# Autodesk Inventor assembly: MIR_HbHand
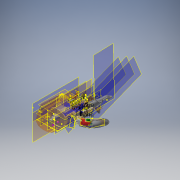
[picture p0: Inventor's stored thumbnail of the model, 180x180]
Saved by Autodesk Inventor 2017 (Build 210142000, 142)
## iProperties
Part Number: MIR_HbHand
Material: 一般
Document SubType Name: Assembly
Designer: sktom
Author: sktom
## Documents named in this file (36)
- D:\OneDrive\CAD\MAJ\hackberry\HACKberry-hardware\3D_69%inlength\Inventor\HbHandForChild\MIR_HbHand.iam
- D:\OneDrive\CAD\MAJ\hackberry\HACKberry-hardware\3D_69%inlength\Inventor\HbHandForChild\MIR_HbPalmBase03ForChild.ipt
- D:\OneDrive\CAD\MAJ\hackberry\HACKberry-hardware\3D_69%inlength\Inventor\HbHandForChild\MIR_bearing_683.ipt
- D:\OneDrive\CAD\MAJ\hackberry\HACKberry-hardware\3D_69%inlength\Inventor\HbHandForChild\HbthumbU02ForChild\MIR_HbthumbU02ForChild.iam
- D:\OneDrive\CAD\MAJ\hackberry\HACKberry-hardware\3D_69%inlength\Inventor\HbHandForChild\HbServoHK282A\MIR_Servo_HK282A_Hone.ipt
- D:\OneDrive\CAD\MAJ\hackberry\HACKberry-hardware\3D_69%inlength\Inventor\HbHandForChild\HbIndexFinger01ForChild\MIR_HbIndexFinger01ForChild.iam
- D:\OneDrive\CAD\MAJ\hackberry\HACKberry-hardware\3D_69%inlength\Inventor\HbHandForChild\HbFinger01ForChild\MIR_HbFinger01ForChild.iam
- D:\OneDrive\CAD\MAJ\hackberry\HACKberry-hardware\3D_69%inlength\Inventor\HbHandForChild\MIR_HbRing-LittleCouplerLink01ForChild.ipt
- D:\OneDrive\CAD\MAJ\hackberry\HACKberry-hardware\3D_69%inlength\Inventor\HbHandForChild\MIR_HbMiddle-RingCouplerLink01ForChild.ipt
- D:\OneDrive\CAD\MAJ\hackberry\HACKberry-hardware\3D_69%inlength\Inventor\HbHandForChild\servo\MIR_Tower Pro 9g Micro Servo SG90.iam
- D:\OneDrive\CAD\MAJ\hackberry\HACKberry-hardware\3D_69%inlength\Inventor\HbHandForChild\MIR_DummyASV-15MG.ipt
- D:\OneDrive\CAD\MAJ\hackberry\HACKberry-hardware\3D_69%inlength\Inventor\HbHandForChild\MIR_HbFingerMainCouplerLink01ForChild.ipt
- D:\OneDrive\CAD\MAJ\hackberry\HACKberry-hardware\3D_69%inlength\Inventor\HbHandForChild\MIR_DummyASV-15MGSingleHorn01.ipt
- D:\OneDrive\CAD\MAJ\hackberry\HACKberry-hardware\3D_69%inlength\Inventor\HbHandForChild\MIR_HbBackCover02ForChild.ipt
- D:\OneDrive\CAD\MAJ\hackberry\HACKberry-hardware\3D_69%inlength\Inventor\HbHandForChild\MIR_Spur Gear (16 teeth).ipt
- D:\OneDrive\CAD\MAJ\hackberry\HACKberry-hardware\3D_69%inlength\Inventor\HbHandForChild\MIR_spacer_2_3_l3.5.ipt
- D:\OneDrive\CAD\MAJ\hackberry\HACKberry-hardware\3D_69%inlength\Inventor\HbHandForChild\MIR_HbServoCover.ipt
- D:\OneDrive\CAD\MAJ\hackberry\HACKberry-hardware\3D_69%inlength\Inventor\HbHandForChild\MIR_HbShaftStopperB04ForChild.ipt
- D:\OneDrive\CAD\MAJ\hackberry\HACKberry-hardware\3D_69%inlength\Inventor\HbHandForChild\MIR_HbShaftStopperA04ForChild.ipt
- D:\OneDrive\CAD\MAJ\hackberry\HACKberry-hardware\3D_69%inlength\Inventor\HbHandForChild\MIR_shaft_phi1.5_l10.ipt
- D:\OneDrive\CAD\MAJ\hackberry\HACKberry-hardware\3D_69%inlength\Inventor\HbHandForChild\MIR_bolt_M2L6.ipt
- D:\OneDrive\CAD\MAJ\hackberry\HACKberry-hardware\3D_69%inlength\Inventor\HbHandForChild\HbCircuit\MIR_HbBoard.ipt
- D:\OneDrive\CAD\MAJ\hackberry\HACKberry-hardware\3D_69%inlength\Inventor\HbHandForChild\MIR_HbPowerLever05ForChild.ipt
- D:\OneDrive\CAD\MAJ\hackberry\HACKberry-hardware\3D_69%inlength\Inventor\HbHandForChild\HbSwitch\MIR_HbFingerLockButton05.ipt
- D:\OneDrive\CAD\MAJ\hackberry\HACKberry-hardware\3D_69%inlength\Inventor\HbHandForChild\HbSwitch\MIR_HbMaxButton05.ipt
- D:\OneDrive\CAD\MAJ\hackberry\HACKberry-hardware\3D_69%inlength\Inventor\HbHandForChild\HbSwitch\MIR_HbMinButton05.ipt
- D:\OneDrive\CAD\MAJ\hackberry\HACKberry-hardware\3D_69%inlength\Inventor\HbHandForChild\HbSwitch\MIR_HbThumbButton05.ipt
- D:\OneDrive\CAD\MAJ\hackberry\HACKberry-hardware\3D_69%inlength\Inventor\HbHandForChild\HbCircuit\MIR_SKRPACE010.ipt
- D:\OneDrive\CAD\MAJ\hackberry\HACKberry-hardware\3D_69%inlength\Inventor\HbHandForChild\HbCircuit\MIR_IS-1250.ipt
- D:\OneDrive\CAD\MAJ\hackberry\HACKberry-hardware\3D_69%inlength\Inventor\HbHandForChild\HbCircuit\MIR_530470310.ipt
- D:\OneDrive\CAD\MAJ\hackberry\HACKberry-hardware\3D_69%inlength\Inventor\HbHandForChild\HbCircuit\MIR_510210300.ipt
- D:\OneDrive\CAD\MAJ\hackberry\HACKberry-hardware\3D_69%inlength\Inventor\HbHandForChild\MIR_bolt_M1.4L6.ipt
- D:\OneDrive\CAD\MAJ\hackberry\HACKberry-hardware\3D_69%inlength\Inventor\HbHandForChild\HbCircuit\MIR_S2B-PH-K-S.ipt
- D:\OneDrive\CAD\MAJ\hackberry\HACKberry-hardware\3D_69%inlength\Inventor\HbHandForChild\HbCircuit\MIR_PHR-2.ipt
- D:\OneDrive\CAD\MAJ\hackberry\HACKberry-hardware\3D_69%inlength\Inventor\HbHandForChild\HbCircuit\MIR_Pololu_A_Star_32U4_Micro.ipt
- D:\OneDrive\CAD\MAJ\hackberry\HACKberry-hardware\3D_69%inlength\Inventor\HbHandForChild\HbCircuit\MIR_S3B-PH-K-S.ipt
## Components (61 placed, 35 different names)
1. MIR_HbPalmBase03ForChild:1 — 挿入:1, 挿入:5, 挿入:4, 挿入:6, 挿入:8, 挿入:7, 挿入:10, 挿入:9, 挿入:12, 挿入:11, 挿入:16, 挿入:15, メイト:3, メイト:2, 挿入:23, 挿入:22, 挿入:32, 挿入:31, 挿入:34, 挿入:33, 挿入:35, 挿入:36, 挿入:37, 挿入:38, 挿入:39, 挿入:41, 挿入:40, フラッシュ:3, メイト:26, メイト:32
2. MIR_bearing_683:1 — 挿入:1, 挿入:2
3. MIR_HbthumbU02ForChild:1 [sub-assembly] — 挿入:2, 挿入:3
4. MIR_Servo_HK282A_Hone:1 — 挿入:5, 挿入:4, 挿入:3, 挿入:53, 挿入:52
5. MIR_HbIndexFinger01ForChild:1 [sub-assembly] — 挿入:6
6. MIR_HbFinger01ForChild:1 [sub-assembly] — 挿入:8, 挿入:7, 挿入:30
7. MIR_HbFinger01ForChild:2 [sub-assembly] — 挿入:10, 挿入:9, 挿入:28, 挿入:29
8. MIR_HbFinger01ForChild:3 [sub-assembly] — 挿入:12, 挿入:11, 挿入:19, 挿入:26, 挿入:27
9. MIR_HbRing-LittleCouplerLink01ForChild:1 — フラッシュ:2, 挿入:46, 挿入:47, 円柱状:6, 円柱状:5
10. MIR_HbMiddle-RingCouplerLink01ForChild:1 — フラッシュ:1, 円柱状:3, 円柱状:4
11. MIR_Tower Pro 9g Micro Servo SG90:1 [sub-assembly] — 挿入:16, 挿入:15, 挿入:24
12. MIR_DummyASV-15MG:1 — メイト:3, メイト:2, 挿入:20
13. MIR_HbFingerMainCouplerLink01ForChild:1 — 挿入:19, 挿入:42, 挿入:43
14. MIR_DummyASV-15MGSingleHorn01:1 — 挿入:42, 挿入:20
15. MIR_HbBackCover02ForChild:1 — 挿入:23, 挿入:22, メイト:5, メイト:4, メイト:7, メイト:6, メイト:11, メイト:10
16. MIR_Spur Gear (16 teeth):1 — 挿入:24
17. MIR_spacer_2_3_l3.5:1 — 挿入:26
18. MIR_spacer_2_3_l3.5:2 — 挿入:43, 挿入:48
19. MIR_spacer_2_3_l3.5:3 — フラッシュ:2, 挿入:27, 円柱状:6
20. MIR_spacer_2_3_l3.5:4 — 挿入:28, 円柱状:5
21. MIR_spacer_2_3_l3.5:5 — フラッシュ:1, 挿入:29, 挿入:45, 円柱状:3
22. MIR_spacer_2_3_l3.5:6 — 挿入:30, 挿入:44, 円柱状:4
23. MIR_HbServoCover:1 — 挿入:32, 挿入:31, 挿入:51, 挿入:50, 挿入:49
24. MIR_HbShaftStopperB04ForChild:1 — 挿入:34
25. MIR_HbShaftStopperA04ForChild:1 — 挿入:33
26. MIR_shaft_phi1.5_l10:1 — 挿入:35
27. MIR_shaft_phi1.5_l10:2 — 挿入:36
28. MIR_shaft_phi1.5_l10:3 — 挿入:37
29. MIR_shaft_phi1.5_l10:4 — 挿入:38
30. MIR_shaft_phi1.5_l10:5 — 挿入:39
31. MIR_shaft_phi1.5_l10:6 — 挿入:41
32. MIR_shaft_phi1.5_l10:7 — 挿入:40
33. MIR_bolt_M2L6:1 — 挿入:44
34. MIR_bolt_M2L6:2 — 挿入:45
35. MIR_bolt_M2L6:3 — 挿入:46
36. MIR_bolt_M2L6:4 — 挿入:47
37. MIR_bolt_M2L6:5 — 挿入:48
38. MIR_HbBoard:1 — フラッシュ:3, メイト:12, メイト:14, メイト:13, メイト:15, メイト:16, フラッシュ:13, メイト:20, メイト:21, メイト:22, フラッシュ:18, メイト:25, フラッシュ:20, メイト:29, フラッシュ:19, メイト:30
39. MIR_HbPowerLever05ForChild:1 — メイト:5, メイト:4
40. MIR_HbFingerLockButton05:1 — メイト:7, メイト:6
41. MIR_HbMaxButton05:1 — メイト:8, フラッシュ:7, フラッシュ:6
42. MIR_HbMinButton05:1 — メイト:11, メイト:10, メイト:8, フラッシュ:7, フラッシュ:6, メイト:9, フラッシュ:5, フラッシュ:4
43. MIR_HbThumbButton05:1 — メイト:9, フラッシュ:5, フラッシュ:4
44. MIR_SKRPACE010:1 — メイト:12, フラッシュ:10, フラッシュ:8, フラッシュ:12
45. MIR_SKRPACE010:2 — フラッシュ:10, フラッシュ:8, メイト:14, フラッシュ:11, フラッシュ:9
46. MIR_SKRPACE010:3 — フラッシュ:12, メイト:13
47. MIR_SKRPACE010:4 — フラッシュ:11, フラッシュ:9, メイト:15
48. MIR_IS-1250:1 — メイト:16
49. MIR_530470310:1 — フラッシュ:13, メイト:20, メイト:19, メイト:18, メイト:17, メイト:23, フラッシュ:14, フラッシュ:15
50. MIR_510210300:1 — メイト:19, メイト:18, メイト:17
51. MIR_530470310:2 — メイト:23, メイト:21, フラッシュ:14, メイト:24
52. MIR_530470310:3 — メイト:24, メイト:22, フラッシュ:15
53. MIR_bolt_M1.4L6:1 — 挿入:51
54. MIR_bolt_M1.4L6:2 — 挿入:50
55. MIR_bolt_M1.4L6:3 — 挿入:49
56. MIR_S2B-PH-K-S:1 — メイト:26, フラッシュ:18, メイト:25, メイト:28, メイト:27
57. MIR_PHR-2:1 — メイト:28, メイト:27
58. MIR_Pololu_A_Star_32U4_Micro:1 — フラッシュ:20, メイト:29, フラッシュ:19
59. MIR_S3B-PH-K-S:1 — メイト:32, メイト:30
60. MIR_bolt_M1.4L6:4 — 挿入:53
61. MIR_bolt_M1.4L6:5 — 挿入:52
## Relationships (99: Insert 47, Mate 31, Flush 17, CylindricalJoint 4)
- 挿入:1 [Insert]: MIR_HbPalmBase03ForChild:1 ↔ MIR_bearing_683:1
- 挿入:2 [Insert]: MIR_bearing_683:1 ↔ MIR_HbthumbU02ForChild:1
- 挿入:5 [Insert]: MIR_HbPalmBase03ForChild:1 ↔ MIR_Servo_HK282A_Hone:1
- 挿入:4 [Insert]: MIR_HbPalmBase03ForChild:1 ↔ MIR_Servo_HK282A_Hone:1
- 挿入:3 [Insert]: MIR_HbthumbU02ForChild:1 ↔ MIR_Servo_HK282A_Hone:1
- 挿入:6 [Insert]: MIR_HbPalmBase03ForChild:1 ↔ MIR_HbIndexFinger01ForChild:1
- 挿入:8 [Insert]: MIR_HbPalmBase03ForChild:1 ↔ MIR_HbFinger01ForChild:1
- 挿入:7 [Insert]: MIR_HbPalmBase03ForChild:1 ↔ MIR_HbFinger01ForChild:1
- 挿入:10 [Insert]: MIR_HbPalmBase03ForChild:1 ↔ MIR_HbFinger01ForChild:2
- 挿入:9 [Insert]: MIR_HbPalmBase03ForChild:1 ↔ MIR_HbFinger01ForChild:2
- 挿入:12 [Insert]: MIR_HbPalmBase03ForChild:1 ↔ MIR_HbFinger01ForChild:3
- 挿入:11 [Insert]: MIR_HbPalmBase03ForChild:1 ↔ MIR_HbFinger01ForChild:3
- 挿入:16 [Insert]: MIR_HbPalmBase03ForChild:1 ↔ MIR_Tower Pro 9g Micro Servo SG90:1
- 挿入:15 [Insert]: MIR_HbPalmBase03ForChild:1 ↔ MIR_Tower Pro 9g Micro Servo SG90:1
- メイト:3 [Mate]: MIR_HbPalmBase03ForChild:1 ↔ MIR_DummyASV-15MG:1
- メイト:2 [Mate]: MIR_HbPalmBase03ForChild:1 ↔ MIR_DummyASV-15MG:1
- 挿入:19 [Insert] (0.1 mm): MIR_HbFinger01ForChild:3 ↔ MIR_HbFingerMainCouplerLink01ForChild:1
- 挿入:42 [Insert]: MIR_HbFingerMainCouplerLink01ForChild:1 ↔ MIR_DummyASV-15MGSingleHorn01:1
- 挿入:20 [Insert]: MIR_DummyASV-15MG:1 ↔ MIR_DummyASV-15MGSingleHorn01:1
- 挿入:23 [Insert]: MIR_HbPalmBase03ForChild:1 ↔ MIR_HbBackCover02ForChild:1
- 挿入:22 [Insert]: MIR_HbPalmBase03ForChild:1 ↔ MIR_HbBackCover02ForChild:1
- 挿入:24 [Insert] (0.8 mm): MIR_Tower Pro 9g Micro Servo SG90:1 ↔ MIR_Spur Gear (16 teeth):1
- 挿入:26 [Insert]: MIR_HbFinger01ForChild:3 ↔ MIR_spacer_2_3_l3.5:1
- 挿入:43 [Insert]: MIR_HbFingerMainCouplerLink01ForChild:1 ↔ MIR_spacer_2_3_l3.5:2
- フラッシュ:2 [Flush]: MIR_HbRing-LittleCouplerLink01ForChild:1 ↔ MIR_spacer_2_3_l3.5:3
- 挿入:27 [Insert]: MIR_HbFinger01ForChild:3 ↔ MIR_spacer_2_3_l3.5:3
- 挿入:28 [Insert]: MIR_HbFinger01ForChild:2 ↔ MIR_spacer_2_3_l3.5:4
- フラッシュ:1 [Flush]: MIR_HbMiddle-RingCouplerLink01ForChild:1 ↔ MIR_spacer_2_3_l3.5:5
- 挿入:29 [Insert]: MIR_HbFinger01ForChild:2 ↔ MIR_spacer_2_3_l3.5:5
- 挿入:30 [Insert]: MIR_HbFinger01ForChild:1 ↔ MIR_spacer_2_3_l3.5:6
- 挿入:32 [Insert]: MIR_HbPalmBase03ForChild:1 ↔ MIR_HbServoCover:1
- 挿入:31 [Insert]: MIR_HbPalmBase03ForChild:1 ↔ MIR_HbServoCover:1
- 挿入:34 [Insert]: MIR_HbPalmBase03ForChild:1 ↔ MIR_HbShaftStopperB04ForChild:1
- 挿入:33 [Insert]: MIR_HbPalmBase03ForChild:1 ↔ MIR_HbShaftStopperA04ForChild:1
- 挿入:35 [Insert]: MIR_HbPalmBase03ForChild:1 ↔ MIR_shaft_phi1.5_l10:1
- 挿入:36 [Insert] (0.5 mm): MIR_HbPalmBase03ForChild:1 ↔ MIR_shaft_phi1.5_l10:2
- 挿入:37 [Insert] (0.3 mm): MIR_HbPalmBase03ForChild:1 ↔ MIR_shaft_phi1.5_l10:3
- 挿入:38 [Insert] (0.3 mm): MIR_HbPalmBase03ForChild:1 ↔ MIR_shaft_phi1.5_l10:4
- 挿入:39 [Insert] (0.5 mm): MIR_HbPalmBase03ForChild:1 ↔ MIR_shaft_phi1.5_l10:5
- 挿入:41 [Insert] (0.5 mm): MIR_HbPalmBase03ForChild:1 ↔ MIR_shaft_phi1.5_l10:6
- 挿入:40 [Insert] (0.5 mm): MIR_HbPalmBase03ForChild:1 ↔ MIR_shaft_phi1.5_l10:7
- 挿入:44 [Insert] (0.3 mm): MIR_spacer_2_3_l3.5:6 ↔ MIR_bolt_M2L6:1
- 挿入:45 [Insert] (0.3 mm): MIR_spacer_2_3_l3.5:5 ↔ MIR_bolt_M2L6:2
- 挿入:46 [Insert] (0.3 mm): MIR_HbRing-LittleCouplerLink01ForChild:1 ↔ MIR_bolt_M2L6:3
- 挿入:47 [Insert] (0.3 mm): MIR_HbRing-LittleCouplerLink01ForChild:1 ↔ MIR_bolt_M2L6:4
- 挿入:48 [Insert] (0.3 mm): MIR_spacer_2_3_l3.5:2 ↔ MIR_bolt_M2L6:5
- フラッシュ:3 [Mate]: MIR_HbPalmBase03ForChild:1 ↔ MIR_HbBoard:1
- メイト:5 [Mate] (0.5 mm): MIR_HbBackCover02ForChild:1 ↔ MIR_HbPowerLever05ForChild:1
- メイト:4 [Mate] (0.3 mm): MIR_HbBackCover02ForChild:1 ↔ MIR_HbPowerLever05ForChild:1
- メイト:7 [Mate] (0.25 mm): MIR_HbBackCover02ForChild:1 ↔ MIR_HbFingerLockButton05:1
- メイト:6 [Mate] (0.5 mm): MIR_HbBackCover02ForChild:1 ↔ MIR_HbFingerLockButton05:1
- メイト:11 [Mate] (0.25 mm): MIR_HbBackCover02ForChild:1 ↔ MIR_HbMinButton05:1
- メイト:10 [Mate] (0.5 mm): MIR_HbBackCover02ForChild:1 ↔ MIR_HbMinButton05:1
- メイト:8 [Mate] (0.25 mm): MIR_HbMaxButton05:1 ↔ MIR_HbMinButton05:1
- フラッシュ:7 [Flush]: MIR_HbMaxButton05:1 ↔ MIR_HbMinButton05:1
- フラッシュ:6 [Flush]: MIR_HbMaxButton05:1 ↔ MIR_HbMinButton05:1
- メイト:9 [Mate] (0.25 mm): MIR_HbMinButton05:1 ↔ MIR_HbThumbButton05:1
- フラッシュ:5 [Flush]: MIR_HbMinButton05:1 ↔ MIR_HbThumbButton05:1
- フラッシュ:4 [Flush]: MIR_HbMinButton05:1 ↔ MIR_HbThumbButton05:1
- メイト:12 [Mate]: MIR_HbBoard:1 ↔ MIR_SKRPACE010:1
- フラッシュ:10 [Flush] (-7.8 mm): MIR_SKRPACE010:1 ↔ MIR_SKRPACE010:2
- フラッシュ:8 [Flush]: MIR_SKRPACE010:1 ↔ MIR_SKRPACE010:2
- メイト:14 [Mate]: MIR_HbBoard:1 ↔ MIR_SKRPACE010:2
- フラッシュ:12 [Flush] (17.911 mm): MIR_SKRPACE010:1 ↔ MIR_SKRPACE010:3
- メイト:13 [Mate]: MIR_HbBoard:1 ↔ MIR_SKRPACE010:3
- フラッシュ:11 [Flush] (-7.8 mm): MIR_SKRPACE010:2 ↔ MIR_SKRPACE010:4
- フラッシュ:9 [Flush]: MIR_SKRPACE010:2 ↔ MIR_SKRPACE010:4
- メイト:15 [Mate]: MIR_HbBoard:1 ↔ MIR_SKRPACE010:4
- メイト:16 [Mate]: MIR_HbBoard:1 ↔ MIR_IS-1250:1
- フラッシュ:13 [Flush] (-0.5 mm): MIR_HbBoard:1 ↔ MIR_530470310:1
- メイト:20 [Mate]: MIR_HbBoard:1 ↔ MIR_530470310:1
- メイト:19 [Mate] (0.4 mm): MIR_530470310:1 ↔ MIR_510210300:1
- メイト:18 [Mate]: MIR_530470310:1 ↔ MIR_510210300:1
- メイト:17 [Mate]: MIR_530470310:1 ↔ MIR_510210300:1
- メイト:23 [Mate] (0.8 mm): MIR_530470310:1 ↔ MIR_530470310:2
- メイト:21 [Mate]: MIR_HbBoard:1 ↔ MIR_530470310:2
- フラッシュ:14 [Flush]: MIR_530470310:1 ↔ MIR_530470310:2
- メイト:24 [Mate] (0.8 mm): MIR_530470310:2 ↔ MIR_530470310:3
- メイト:22 [Mate]: MIR_HbBoard:1 ↔ MIR_530470310:3
- フラッシュ:15 [Flush]: MIR_530470310:1 ↔ MIR_530470310:3
- 挿入:51 [Insert]: MIR_HbServoCover:1 ↔ MIR_bolt_M1.4L6:1
- 挿入:50 [Insert]: MIR_HbServoCover:1 ↔ MIR_bolt_M1.4L6:2
- 挿入:49 [Insert]: MIR_HbServoCover:1 ↔ MIR_bolt_M1.4L6:3
- メイト:26 [Mate] (0.5 mm): MIR_HbPalmBase03ForChild:1 ↔ MIR_S2B-PH-K-S:1
- フラッシュ:18 [Flush] (2 mm): MIR_HbBoard:1 ↔ MIR_S2B-PH-K-S:1
- メイト:25 [Mate]: MIR_HbBoard:1 ↔ MIR_S2B-PH-K-S:1
- メイト:28 [Mate]: MIR_S2B-PH-K-S:1 ↔ MIR_PHR-2:1
- メイト:27 [Mate]: MIR_S2B-PH-K-S:1 ↔ MIR_PHR-2:1
- フラッシュ:20 [Flush]: MIR_HbBoard:1 ↔ MIR_Pololu_A_Star_32U4_Micro:1
- メイト:29 [Mate] (2 mm): MIR_HbBoard:1 ↔ MIR_Pololu_A_Star_32U4_Micro:1
- フラッシュ:19 [Flush] (-3 mm): MIR_HbBoard:1 ↔ MIR_Pololu_A_Star_32U4_Micro:1
- メイト:32 [Mate] (-2 mm): MIR_HbPalmBase03ForChild:1 ↔ MIR_S3B-PH-K-S:1
- メイト:30 [Mate]: MIR_HbBoard:1 ↔ MIR_S3B-PH-K-S:1
- 挿入:53 [Insert]: MIR_Servo_HK282A_Hone:1 ↔ MIR_bolt_M1.4L6:4
- 挿入:52 [Insert]: MIR_Servo_HK282A_Hone:1 ↔ MIR_bolt_M1.4L6:5
- 円柱状:6 [CylindricalJoint]: MIR_HbRing-LittleCouplerLink01ForChild:1 ↔ MIR_spacer_2_3_l3.5:3
- 円柱状:5 [CylindricalJoint]: MIR_HbRing-LittleCouplerLink01ForChild:1 ↔ MIR_spacer_2_3_l3.5:4
- 円柱状:3 [CylindricalJoint]: MIR_HbMiddle-RingCouplerLink01ForChild:1 ↔ MIR_spacer_2_3_l3.5:5
- 円柱状:4 [CylindricalJoint]: MIR_HbMiddle-RingCouplerLink01ForChild:1 ↔ MIR_spacer_2_3_l3.5:6
